# Autodesk Inventor assembly: Glovebox_With_Ports
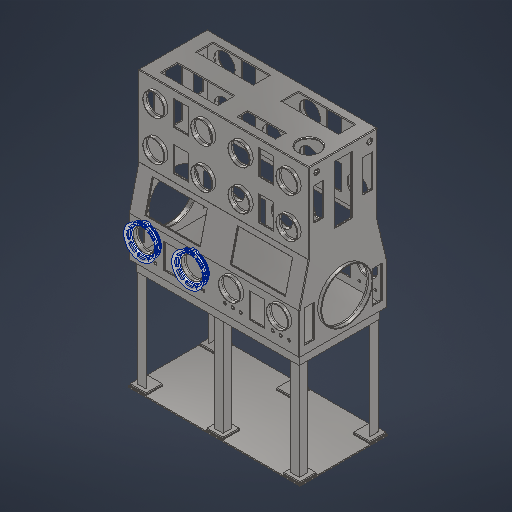
[picture p0: Inventor's stored thumbnail of the model, 512x512]
Saved by Autodesk Inventor 2026.1 (Build 301233000, 233)
## iProperties
Created: 2025-08-29
Part Number: Glovebox_With_Ports
Document SubType Name: Assembly
Designer: alex
Author: alex
## Documents named in this file (3)
- E:\Shared\LANL-Glovebox-Closure-Mechanism\Glovebox_With_Ports.iam
- E:\Shared\LANL-Glovebox-Closure-Mechanism\Glovebox 3D Model Updated.ipt
- E:\Shared\LANL-Glovebox-Closure-Mechanism\Glove_ring.ipt
## Components (3 placed, 2 different names)
1. Glovebox 3D Model Updated:1 — Mate:1, Mate:2, Insert:1, Insert:2
2. Glove_ring:1 — Mate:1, Insert:2
3. Glove_ring:2 — Mate:2, Insert:1
## Relationships (4: Mate 2, Insert 2)
- Mate:1: Glovebox 3D Model Updated:1 ↔ Glove_ring:1
- Mate:2: Glovebox 3D Model Updated:1 ↔ Glove_ring:2
- Insert:1: Glovebox 3D Model Updated:1 ↔ Glove_ring:2
- Insert:2: Glovebox 3D Model Updated:1 ↔ Glove_ring:1
